# Autodesk Inventor assembly: sim_cyc_nema17
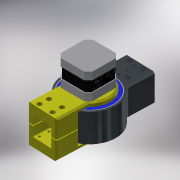
[picture p0: Inventor's stored thumbnail of the model, 180x180]
Saved by Autodesk Inventor 2020.3 (Build 243373000, 373)
## iProperties
Created: 2021-02-24
Part Number: sim_cyc_nema17
Document SubType Name: Assembly
Designer: paulg
Author: paulg
## Documents named in this file (20)
- F:\UQ Engineering\2021 ~ 5th Year\Semester 2\METR4911-THESIS\FarmBot CAD\FarmBotV1\CycloidalJoint\simple_cyc_nema17\sim_cyc_nema17.iam
- F:\UQ Engineering\2021 ~ 5th Year\Semester 2\METR4911-THESIS\FarmBot CAD\FarmBotV1\CycloidalJoint\simple_cyc_nema17\ecc_shaft.ipt
- F:\UQ Engineering\2021 ~ 5th Year\Semester 2\METR4911-THESIS\FarmBot CAD\FarmBotV1\CycloidalJoint\Cycloid CAD\65x50x7 bearing.ipt
- F:\UQ Engineering\2021 ~ 5th Year\Semester 2\METR4911-THESIS\FarmBot CAD\FarmBotV1\CycloidalJoint\simple_cyc_nema17\Motor_paso.ipt
- F:\UQ Engineering\2021 ~ 5th Year\Semester 2\METR4911-THESIS\FarmBot CAD\FarmBotV1\CycloidalJoint\simple_cyc_nema17\base_stepper.ipt
- F:\UQ Engineering\2021 ~ 5th Year\Semester 2\METR4911-THESIS\FarmBot CAD\FarmBotV1\CycloidalJoint\simple_cyc_nema17\output_housing.ipt
- F:\UQ Engineering\2021 ~ 5th Year\Semester 2\METR4911-THESIS\FarmBot CAD\FarmBotV1\CycloidalJoint\Cycloid CAD\18x12x4 bearing.ipt
- F:\UQ Engineering\2021 ~ 5th Year\Semester 2\METR4911-THESIS\FarmBot CAD\FarmBotV1\CycloidalJoint\bldc_capstan\27x20x4 bearing.ipt
- F:\UQ Engineering\2021 ~ 5th Year\Semester 2\METR4911-THESIS\FarmBot CAD\FarmBotV1\CycloidalJoint\simple_cyc_nema17\base_top.ipt
- F:\UQ Engineering\2021 ~ 5th Year\Semester 2\METR4911-THESIS\FarmBot CAD\FarmBotV1\CycloidalJoint\simple_cyc_nema17\Main_equation_step_simple.ipt
- F:\UQ Engineering\2021 ~ 5th Year\Semester 2\METR4911-THESIS\FarmBot CAD\FarmBotV1\CycloidalJoint\simple_cyc_nema17\Main_equation_step_simple_upper.ipt
- F:\UQ Engineering\2021 ~ 5th Year\Semester 2\METR4911-THESIS\FarmBot CAD\FarmBotV1\CycloidalJoint\simple_cyc_nema17\bottom_clip.ipt
- F:\UQ Engineering\2021 ~ 5th Year\Semester 2\METR4911-THESIS\FarmBot CAD\FarmBotV1\CycloidalJoint\simple_cyc_nema17\top_clip.ipt
- F:\UQ Engineering\2021 ~ 5th Year\Semester 2\METR4911-THESIS\FarmBot CAD\FarmBotV1\CycloidalJoint\simple_cyc_nema17\m3 nut.ipt
- F:\UQ Engineering\2021 ~ 5th Year\Semester 2\METR4911-THESIS\FarmBot CAD\FarmBotV1\CycloidalJoint\simple_cyc_nema17\m3_setscrew.ipt
- F:\UQ Engineering\2021 ~ 5th Year\Semester 2\METR4911-THESIS\FarmBot CAD\FarmBotV1\CycloidalJoint\Cycloid CAD\15x10x4 bearing.ipt
- F:\UQ Engineering\2021 ~ 5th Year\Semester 2\METR4911-THESIS\FarmBot CAD\FarmBotV1\CycloidalJoint\Cycloid CAD\mag_6mm.iam
- F:\UQ Engineering\2021 ~ 5th Year\Semester 2\METR4911-THESIS\FarmBot CAD\FarmBotV1\CycloidalJoint\Cycloid CAD\8x5x2.5 bearing.ipt
- F:\UQ Engineering\2021 ~ 5th Year\Semester 2\METR4911-THESIS\FarmBot CAD\FarmBotV1\CycloidalJoint\old-new-cycloidal\3mm_pin.ipt
- F:\UQ Engineering\2021 ~ 5th Year\Semester 2\METR4911-THESIS\FarmBot CAD\FarmBotV1\CycloidalJoint\old-new-cycloidal\Parameters_stepper_simple.xlsx
## Components (43 placed, 18 different names)
1. ecc_shaft:1 — Insert:5, Insert:7, Insert:8, Mate:2, Insert:14, Mate:3, Insert:16, Insert:17, Insert:18, Insert:21, Insert:29, Insert:47
2. 65x50x7 bearing:1 — Insert:2, Insert:48
3. Motor_paso:1 — Mate:1, Insert:47
4. base_stepper:1 — Mate:1, Insert:2, Flush:1, Insert:39, Insert:40, Insert:41, Insert:42, Insert:43, Insert:44, Insert:45, Insert:46
5. output_housing:1 — Insert:9, Insert:48
6. 18x12x4 bearing:1 — Insert:8, Insert:12
7. 18x12x4 bearing:2 — Insert:7
8. 27x20x4 bearing:1 — Insert:5
9. 27x20x4 bearing:2 — Insert:20, Insert:29
10. base_top:1 — Insert:10, Flush:1
11. 65x50x7 bearing:2 — Insert:9, Insert:10
12. Main_equation_step_simple_upper:1 — Insert:12, Insert:31, Insert:32, Insert:33, Insert:34, Insert:35, Insert:36, Insert:37, Insert:38
13. bottom_clip:1 — Mate:2, Insert:14
14. top_clip:1 — Mate:3, Insert:16, Insert:19
15. m3 nut:1 — Insert:17
16. m3_setscrew:1 — Insert:18
17. 15x10x4 bearing:1 — Insert:19
18. Main_equation_step_simple:1 — Insert:20, Insert:22, Insert:23, Insert:24, Insert:25, Insert:26, Insert:27, Insert:28, Insert:30
19. mag_6mm:1 [sub-assembly] — Insert:21
20. 8x5x2.5 bearing:1 — Insert:22
21. 8x5x2.5 bearing:2 — Insert:36
22. 8x5x2.5 bearing:3 — Insert:35
23. 8x5x2.5 bearing:4 — Insert:34, Tangent:1
24. 8x5x2.5 bearing:5 — Insert:32
25. 8x5x2.5 bearing:6 — Insert:30, Tangent:2
26. 8x5x2.5 bearing:7 — Insert:31
27. 8x5x2.5 bearing:8 — Insert:23
28. 8x5x2.5 bearing:9 — Insert:24
29. 8x5x2.5 bearing:10 — Insert:25
30. 8x5x2.5 bearing:11 — Insert:28
31. 8x5x2.5 bearing:12 — Insert:37
32. 8x5x2.5 bearing:14 — Insert:33
33. 8x5x2.5 bearing:19 — Insert:27
34. 8x5x2.5 bearing:20 — Insert:26
35. 8x5x2.5 bearing:21 — Insert:38
36. 3mm_pin:2 — Insert:41
37. 3mm_pin:4 — Insert:46, Tangent:1, Tangent:2
38. 3mm_pin:5 — Insert:44
39. 3mm_pin:6 — Insert:42
40. 3mm_pin:7 — Insert:39
41. 3mm_pin:8 — Insert:40
42. 3mm_pin:9 — Insert:45
43. 3mm_pin:10 — Insert:43
## Relationships (47: Insert 41, Mate 3, Tangent 2, Flush 1)
- Mate:1: Motor_paso:1 ↔ base_stepper:1
- Insert:2: 65x50x7 bearing:1 ↔ base_stepper:1
- Insert:5: ecc_shaft:1 ↔ 27x20x4 bearing:1
- Insert:7: ecc_shaft:1 ↔ 18x12x4 bearing:2
- Insert:8: ecc_shaft:1 ↔ 18x12x4 bearing:1
- Insert:9: output_housing:1 ↔ 65x50x7 bearing:2
- Insert:10: base_top:1 ↔ 65x50x7 bearing:2
- Flush:1: base_stepper:1 ↔ base_top:1
- Insert:12: 18x12x4 bearing:1 ↔ Main_equation_step_simple_upper:1
- Mate:2: ecc_shaft:1 ↔ bottom_clip:1
- Insert:14: ecc_shaft:1 ↔ bottom_clip:1
- Mate:3: ecc_shaft:1 ↔ top_clip:1
- Insert:16: ecc_shaft:1 ↔ top_clip:1
- Insert:17: ecc_shaft:1 ↔ m3 nut:1
- Insert:18 (-3 mm): ecc_shaft:1 ↔ m3_setscrew:1
- Insert:19: top_clip:1 ↔ 15x10x4 bearing:1
- Insert:20: 27x20x4 bearing:2 ↔ Main_equation_step_simple:1
- Insert:21: ecc_shaft:1 ↔ mag_6mm:1
- Insert:22: Main_equation_step_simple:1 ↔ 8x5x2.5 bearing:1
- Insert:23: Main_equation_step_simple:1 ↔ 8x5x2.5 bearing:8
- Insert:24: Main_equation_step_simple:1 ↔ 8x5x2.5 bearing:9
- Insert:25: Main_equation_step_simple:1 ↔ 8x5x2.5 bearing:10
- Insert:26: Main_equation_step_simple:1 ↔ 8x5x2.5 bearing:20
- Insert:27: Main_equation_step_simple:1 ↔ 8x5x2.5 bearing:19
- Insert:28: Main_equation_step_simple:1 ↔ 8x5x2.5 bearing:11
- Insert:29: ecc_shaft:1 ↔ 27x20x4 bearing:2
- Insert:30: Main_equation_step_simple:1 ↔ 8x5x2.5 bearing:6
- Insert:31: Main_equation_step_simple_upper:1 ↔ 8x5x2.5 bearing:7
- Insert:32: Main_equation_step_simple_upper:1 ↔ 8x5x2.5 bearing:5
- Insert:33: Main_equation_step_simple_upper:1 ↔ 8x5x2.5 bearing:14
- Insert:34: Main_equation_step_simple_upper:1 ↔ 8x5x2.5 bearing:4
- Insert:35: Main_equation_step_simple_upper:1 ↔ 8x5x2.5 bearing:3
- Insert:36: Main_equation_step_simple_upper:1 ↔ 8x5x2.5 bearing:2
- Insert:37: Main_equation_step_simple_upper:1 ↔ 8x5x2.5 bearing:12
- Insert:38: Main_equation_step_simple_upper:1 ↔ 8x5x2.5 bearing:21
- Insert:39: base_stepper:1 ↔ 3mm_pin:7
- Insert:40: base_stepper:1 ↔ 3mm_pin:8
- Insert:41: base_stepper:1 ↔ 3mm_pin:2
- Insert:42: base_stepper:1 ↔ 3mm_pin:6
- Insert:43: base_stepper:1 ↔ 3mm_pin:10
- Insert:44: base_stepper:1 ↔ 3mm_pin:5
- Insert:45: base_stepper:1 ↔ 3mm_pin:9
- Insert:46: base_stepper:1 ↔ 3mm_pin:4
- Insert:47 (1 mm): ecc_shaft:1 ↔ Motor_paso:1
- Tangent:1: 8x5x2.5 bearing:4 ↔ 3mm_pin:4
- Tangent:2: 8x5x2.5 bearing:6 ↔ 3mm_pin:4
- Insert:48: 65x50x7 bearing:1 ↔ output_housing:1
## Named parameters: N_ = 25, E_ = 1 mm, Rr_ = 2 mm, R_ = 31.5 mm
